# Autodesk Inventor assembly: RoundyMotor
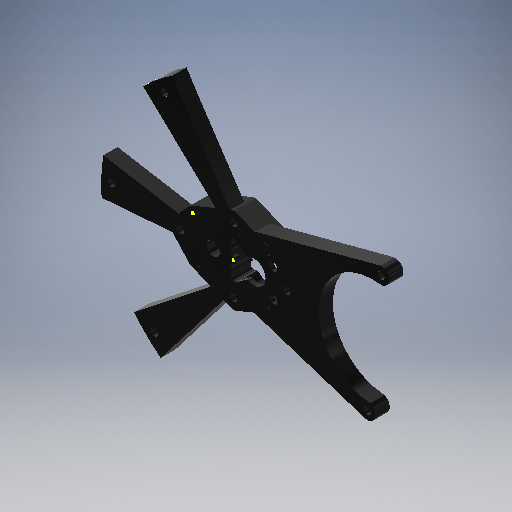
[picture p0: Inventor's stored thumbnail of the model, 512x512]
Saved by Autodesk Inventor 2026.1 (Build 301233000, 233)
## iProperties
Created: 2025-10-13
Part Number: RoundyMotor
Document SubType Name: Assembly
Designer: Teddy
Author: Teddy
## Documents named in this file (3)
- C:\Users\Teddy\Desktop\VexCAD\15InVEX\RoundyMotor.iam
- C:\Users\Teddy\Desktop\VexCAD\15FEBOY\MotorCap.ipt
- C:\Users\Teddy\Desktop\VexCAD\15InVEX\MotorConnectionRoundyBit.ipt
## Components (2 placed, 2 different names)
1. MotorCap:1 — Mate:1, Flush:1, Mate:2
2. MotorConnectionRoundyBit:1 — Mate:1, Flush:1, Mate:2
## Relationships (3: Mate 2, Flush 1)
- Mate:1 (-1.27 mm): MotorCap:1 ↔ MotorConnectionRoundyBit:1
- Flush:1: MotorCap:1 ↔ MotorConnectionRoundyBit:1
- Mate:2 (-1.27 mm): MotorCap:1 ↔ MotorConnectionRoundyBit:1
